# Autodesk Inventor assembly: Сборка_редуктор+муфта
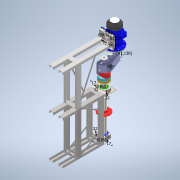
[picture p0: Inventor's stored thumbnail of the model, 180x180]
Saved by Autodesk Inventor 2021 (Build 250183000, 183)
## iProperties
Created: 2023-04-27
Part Number: Сборка_редуктор+муфта
Document SubType Name: Assembly
Designer: gdevc
Mass: 103016 g
Surface Area: 49542.2 cm^2
Volume: 25213.8 cm^3
Density: 4.08568 g/cm^3
Author: gdevc
## Documents named in this file (5)
- C:\Users\gdevc\OneDrive\Рабочий стол\Курсач\DetaliMashine\Новая папка\Сборка_редуктора+муфта\Сборка_редуктор+муфта.iam
- C:\Users\gdevc\OneDrive\Рабочий стол\Курсач\DetaliMashine\Новая папка\Сборка_новая.iam
- C:\Users\gdevc\OneDrive\Рабочий стол\Курсач\DetaliMashine\Новая папка\Муфта в сборе.iam
- C:\Users\gdevc\OneDrive\Рабочий стол\Курсач\DetaliMashine\Новая папка\Приводной валл\Сборка вала.iam
- C:\Users\gdevc\OneDrive\Рабочий стол\Курсач\DetaliMashine\Новая папка\Рама\Рама.iam
## Components (4 placed, 4 different names)
1. Сборка_новая:1 [sub-assembly] — Совмещение:1, Совмещение:2
2. Муфта в сборе:1 [sub-assembly] — Совмещение:1, Угол:1, Совмещение:2, Совмещение:3
3. Сборка вала:1 [sub-assembly] — Совмещение:3, Угол:2, Совмещение:4, Заподлицо:1, Заподлицо:2
4. Рама:1 [sub-assembly] — Угол:3, Угол:4, Совмещение:4, Заподлицо:1, Заподлицо:2
## Relationships (10: Mate 4, Angle 4, Flush 2)
- Совмещение:1 [Mate]: Сборка_новая:1 ↔ Муфта в сборе:1
- Угол:1 [Angle] (180 deg): Муфта в сборе:1
- Совмещение:2 [Mate] (8.8 mm): Сборка_новая:1 ↔ Муфта в сборе:1
- Совмещение:3 [Mate]: Муфта в сборе:1 ↔ Сборка вала:1
- Угол:2 [Angle] (0 deg): Сборка вала:1
- Угол:3 [Angle] (0 deg): Рама:1
- Угол:4 [Angle] (0 deg): Рама:1
- Совмещение:4 [Mate]: Сборка вала:1 ↔ Рама:1
- Заподлицо:1 [Flush]: Сборка вала:1 ↔ Рама:1
- Заподлицо:2 [Flush]: Сборка вала:1 ↔ Рама:1
